# Autodesk Inventor assembly: hegnspæl omvendt
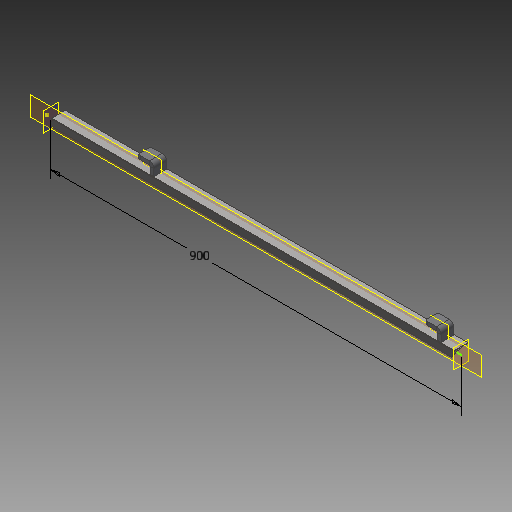
[picture p0: Inventor's stored thumbnail of the model, 512x512]
Saved by Autodesk Inventor 2018 (Build 220112000, 112)
## iProperties
Created: 2019-09-30
Part Number: hegnspæl omvendt
Document SubType Name: Assembly
Designer: gust3763
Mass: 1821.47 g
Surface Area: 1100.09 cm^2
Volume: 232.034 cm^3
Density: 7.85 g/cm^3
_SolveAssemblyDoc: Frame Generator Solve Assembly
_Version: 15.0.0
Author: gust3763
## Documents named in this file (6)
- Z:\trappe\hegn\hegnspæl omvendt.iam
- hegnspæl omvendt.iam
- Z:\trappe\hegn\t-profil.ipt
- Z:\trappe\hegn\t-profil\Frame\Frame0002.iam
- Z:\trappe\hegn\hage.ipt
- Z:\trappe\trappe.xlsx
## Components (4 placed, 3 different names)
1. t-profil:1
2. Frame0002:1 [sub-assembly] — Mate:1, Mate:2, Flush:1, Flush:2, Flush:4, Mate:3, Angle:1, Mate:4, Angle:2, Mate:5, Angle:3
3. hage:1 — Mate:1, Flush:2, Flush:3
4. hage:2 — Mate:2, Flush:1, Flush:3, Flush:4
## Relationships (12: Mate 5, Flush 4, Angle 3)
- Mate:1: Frame0002:1 ↔ hage:1
- Mate:2: Frame0002:1 ↔ hage:2
- Flush:1 (1 mm): Frame0002:1 ↔ hage:2
- Flush:2 (1 mm): Frame0002:1 ↔ hage:1
- Flush:3 (-630 mm): hage:1 ↔ hage:2
- Flush:4 (30 mm): Frame0002:1 ↔ hage:2
- Mate:3: Frame0002:1
- Angle:1 (0 deg): Frame0002:1
- Mate:4: Frame0002:1
- Angle:2 (0 deg): Frame0002:1
- Mate:5: Frame0002:1
- Angle:3 (0 deg): Frame0002:1
## Named parameters: trappevinkel = 34.3 deg, trappestifter_dia = 25 mm, trappestifter_huldia = 25.8 mm, trappestifter_skraa_huldia = 26.6 mm, trappestifter_laengde = 228 mm, perforeringsbredde = 6 mm, perforeringshulprocent = 80 mm, perforeringshullaengde = 62.8 mm, perforeringshullaengde_top = 61 mm, perforeringshullaengde_bund = 61.6 mm, perforeringsoffset = 8 mm, perforeringsoffset_top = 8 mm, perforeringsoffset_bund = 8 mm, laskehul_dia = 13 mm, haandfang_offset_fra_top = 90 mm, balusterhul_udvidelse = 1 mm, pladetykkelse = 3 mm
